# Autodesk Inventor assembly: AssemblyPeleCarotte
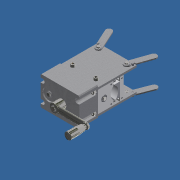
[picture p0: Inventor's stored thumbnail of the model, 180x180]
Saved by Autodesk Inventor 2018 (Build 220112000, 112)
## iProperties
Created: 2022-02-21
Part Number: AssemblyPeleCarotte
Document SubType Name: Assembly
Designer: Nathann
Mass: 1273.76 g
Surface Area: 2275.54 cm^2
Volume: 544.926 cm^3
Density: 2.3375 g/cm^3
Author: Nathann
## Documents named in this file (28)
- C:\Users\Nathann\OneDrive\Objet3D\EPFLEplucheCarrote\V9\AssemblyPeleCarotte-SURFACE-NAT.iam
- C:\Users\Nathann\OneDrive\Objet3D\EPFLEplucheCarrote\V9\Carrot_Peeler_Blade.ipt
- C:\Users\Nathann\OneDrive\Objet3D\EPFLEplucheCarrote\V9\GuideCarotte.ipt
- C:\Users\Nathann\OneDrive\Objet3D\EPFLEplucheCarrote\V9\PlaqueGuideBlocLame.ipt
- C:\Users\Nathann\OneDrive\Objet3D\EPFLEplucheCarrote\V9\2662N415_20DegreePressureAnglePlasticGear.ipt
- C:\Users\Nathann\OneDrive\Objet3D\EPFLEplucheCarrote\V9\2810N4_PlasticMiterGear.ipt
- C:\Users\Nathann\OneDrive\Objet3D\EPFLEplucheCarrote\V9\2662N435_20DegreePressureAnglePlasticGear.ipt
- C:\Users\Nathann\OneDrive\Objet3D\EPFLEplucheCarrote\V9\JointTorique.ipt
- C:\Users\Nathann\Documents\Inventor\Content Center Files\R2018\en-US\SS-ISO 4762\ISO 4762 - M6 x 12SS-ISO.ipt
- C:\Users\Nathann\OneDrive\Objet3D\EPFLEplucheCarrote\V9\Jambe.ipt
- C:\Users\Nathann\OneDrive\Objet3D\EPFLEplucheCarrote\V9\57785K318_Food Industry Dry-Running Sleeve Bearing.ipt
- C:\Users\Nathann\OneDrive\Objet3D\EPFLEplucheCarrote\V9\57785K314_Food Industry Dry-Running Sleeve Bearing-MINOUCHE.ipt
- C:\Users\Nathann\OneDrive\Objet3D\EPFLEplucheCarrote\V9\Roller.ipt
- C:\Users\Nathann\OneDrive\Objet3D\EPFLEplucheCarrote\V9\CarterEngrennage.ipt
- C:\Users\Nathann\OneDrive\Objet3D\EPFLEplucheCarrote\V9\AxeVerticalCaptif.ipt
- C:\Users\Nathann\OneDrive\Objet3D\EPFLEplucheCarrote\V9\AxeVerticalManivelle.ipt
- C:\Users\Nathann\OneDrive\Objet3D\EPFLEplucheCarrote\V9\AxeJambe.ipt
- C:\Users\Nathann\OneDrive\Objet3D\EPFLEplucheCarrote\V9\AxeHorizontalRoller.ipt
- C:\Users\Nathann\OneDrive\Objet3D\EPFLEplucheCarrote\V9\92605A528_Stainless Steel Flat-Tip Set Screw.ipt
- C:\Users\Nathann\OneDrive\Objet3D\EPFLEplucheCarrote\V9\6545N13_303 Stainless Steel Unthreaded Through-Hole Crank Handle.ipt
- C:\Users\Nathann\OneDrive\Objet3D\EPFLEplucheCarrote\V9\2977N13_Rounded Machine Key.ipt
- C:\Users\Nathann\OneDrive\Objet3D\EPFLEplucheCarrote\V9\2977N12_Rounded Machine Key.ipt
- C:\Users\Nathann\OneDrive\Objet3D\EPFLEplucheCarrote\V9\1942N55_Corrosion-Resistant Extension Springs with Hook Ends.ipt
- C:\Users\Nathann\OneDrive\Objet3D\EPFLEplucheCarrote\V9\SupportGuideCarotte.ipt
- C:\Users\Nathann\OneDrive\Objet3D\EPFLEplucheCarrote\V9\93600A511_316 Stainless Steel Dowel Pin.ipt
- C:\Users\Nathann\OneDrive\Objet3D\EPFLEplucheCarrote\V9\93600A531_316 Stainless Steel Dowel Pin.ipt
- C:\Users\Nathann\OneDrive\Objet3D\EPFLEplucheCarrote\V9\98317A224_Side-Mount External Retaining Ring.ipt
- C:\Users\Nathann\OneDrive\Objet3D\EPFLEplucheCarrote\V9\CarterRouleau.ipt
## Components (86 placed, 27 different names)
1. CarterRouleau:1 — Insert:163, Insert:164, Insert:165, Insert:166, Insert:167, Insert:168, Mate:11, Insert:169, Insert:170, Insert:175, Insert:176, Insert:177, Insert:179
2. CarterEngrennage:1 — Insert:21, Insert:22, Insert:23, Insert:24, Insert:85, Insert:93, Insert:97, Insert:98, Insert:167, Insert:168
3. GuideCarotte:1 — Insert:182
4. Carrot_Peeler_Blade:3
5. PlaqueGuideBlocLame:1 — Insert:18, Insert:20, Insert:42, Insert:52, Insert:53, Insert:61, Insert:71, Mate:10, Flush:1, Insert:147, Insert:148, Mate:11, Insert:169, Insert:170, Insert:171, Insert:172
6. PlaqueGuideBlocLame:3 — Insert:104, Insert:119, Insert:120, Insert:145, Insert:146, Insert:177, Insert:178, Insert:179, Insert:180, Insert:181
7. 2662N415_20DegreePressureAnglePlasticGear:1 — Insert:89, Rotation:10, Mate:20, Insert:189, Rotation:17
8. 2810N4_PlasticMiterGear:1 — Insert:83, Mate:19
9. 2810N4_PlasticMiterGear:2 — Insert:89, Rotation:17
10. 2662N435_20DegreePressureAnglePlasticGear:1 — Insert:100, Rotation:2
11. Roller:1 — Insert:82, Insert:83, Mate:18
12. AxeVerticalCaptif:1 — Rotation:4, Rotation:10, Mate:6, Mate:7, Rotation:16, Insert:150, Insert:152, Insert:174, Insert:186, Insert:187, Mate:21, Insert:188
13. AxeVerticalManivelle:1 — Rotation:2, Rotation:4, Mate:2, Mate:3, Mate:4, Mate:5, Rotation:15, Insert:149, Insert:151, Mate:12, Mate:13, Insert:183, Insert:190
14. AxeHorizontalRoller:1 — Insert:81, Mate:8, Mate:9, Rotation:16, Insert:153, Insert:154, Mate:14, Mate:15, Mate:16, Mate:17, Insert:184, Insert:185
15. AxeJambe:1 — Insert:157, Insert:181
16. AxeJambe:2 — Insert:52, Insert:155
17. AxeJambe:3 — Insert:53, Insert:156
18. AxeJambe:4 — Insert:158, Insert:180
19. Jambe:1 — Insert:42, Insert:61
20. Jambe:3 — Insert:120
21. Jambe:4 — Insert:119
22. Jambe:5 — Insert:71
23. 57785K318_Food Industry Dry-Running Sleeve Bearing:1 — Insert:93, Insert:138
24. 57785K318_Food Industry Dry-Running Sleeve Bearing:2 — Insert:98, Insert:100
25. 57785K314_Food Industry Dry-Running Sleeve Bearing-MINOUCHE:1 — Insert:82, Insert:176
26. 57785K314_Food Industry Dry-Running Sleeve Bearing-MINOUCHE:2
27. 57785K314_Food Industry Dry-Running Sleeve Bearing-MINOUCHE:4 — Insert:97, Insert:189
28. 57785K314_Food Industry Dry-Running Sleeve Bearing-MINOUCHE:5 — Insert:81, Insert:175, Insert:185
29. 57785K314_Food Industry Dry-Running Sleeve Bearing-MINOUCHE:6 — Insert:85, Insert:174, Insert:187
30. SupportGuideCarotte:1 — Insert:141, Insert:142, Mate:10, Flush:1, Insert:159, Insert:160, Insert:161, Insert:162, Insert:182
31. 6545N13_303 Stainless Steel Unthreaded Through-Hole Crank Handle:1 — Insert:138, Rotation:15, Insert:183
32. JointTorique:10
33. JointTorique:11
34. JointTorique:12
35. JointTorique:13
36. JointTorique:14
37. JointTorique:15
38. JointTorique:16
39. JointTorique:17
40. 92605A528_Stainless Steel Flat-Tip Set Screw:1
41. 92605A528_Stainless Steel Flat-Tip Set Screw:2
42. 2977N13_Rounded Machine Key:1 — Mate:4, Mate:5, Insert:190
43. 2977N13_Rounded Machine Key:2 — Mate:2, Mate:3, Mate:12, Mate:13
44. 2977N12_Rounded Machine Key:2 — Mate:6, Mate:7, Mate:20, Mate:21, Insert:188
45. 2977N12_Rounded Machine Key:4 — Mate:8, Mate:9, Mate:14, Mate:16
46. 1942N55_Corrosion-Resistant Extension Springs with Hook Ends:1
47. 1942N55_Corrosion-Resistant Extension Springs with Hook Ends:2
48. 1942N55_Corrosion-Resistant Extension Springs with Hook Ends:3
49. 1942N55_Corrosion-Resistant Extension Springs with Hook Ends:4
50. 1942N55_Corrosion-Resistant Extension Springs with Hook Ends:5
51. 1942N55_Corrosion-Resistant Extension Springs with Hook Ends:6
52. 1942N55_Corrosion-Resistant Extension Springs with Hook Ends:7
53. 1942N55_Corrosion-Resistant Extension Springs with Hook Ends:8
54. 93600A511_316 Stainless Steel Dowel Pin:1 — Insert:146
55. 93600A531_316 Stainless Steel Dowel Pin:1 — Insert:163
56. 93600A511_316 Stainless Steel Dowel Pin:2 — Insert:145
57. 93600A511_316 Stainless Steel Dowel Pin:3 — Insert:147
58. 93600A511_316 Stainless Steel Dowel Pin:4 — Insert:148
59. 93600A531_316 Stainless Steel Dowel Pin:2 — Insert:164
60. 93600A531_316 Stainless Steel Dowel Pin:3 — Insert:165
61. 93600A531_316 Stainless Steel Dowel Pin:4 — Insert:166
62. 93600A531_316 Stainless Steel Dowel Pin:5 — Insert:162
63. 93600A531_316 Stainless Steel Dowel Pin:6 — Insert:161
64. 93600A531_316 Stainless Steel Dowel Pin:7 — Insert:159
65. 93600A531_316 Stainless Steel Dowel Pin:8 — Insert:160
66. 98317A224_Side-Mount External Retaining Ring:1 — Insert:149
67. 98317A224_Side-Mount External Retaining Ring:2 — Insert:150, Insert:186
68. 98317A224_Side-Mount External Retaining Ring:3 — Insert:154, Insert:184
69. 98317A224_Side-Mount External Retaining Ring:4 — Insert:151
70. 98317A224_Side-Mount External Retaining Ring:5 — Insert:152
71. 98317A224_Side-Mount External Retaining Ring:6 — Insert:153
72. 98317A224_Side-Mount External Retaining Ring:7 — Insert:157
73. 98317A224_Side-Mount External Retaining Ring:8 — Insert:158
74. 98317A224_Side-Mount External Retaining Ring:9 — Insert:156
75. 98317A224_Side-Mount External Retaining Ring:10 — Insert:155
76. SS ISO 4762 M6 x 12:4 — Insert:141
77. SS ISO 4762 M6 x 12:5 — Insert:178
78. SS ISO 4762 M6 x 12:6 — Insert:104
79. SS ISO 4762 M6 x 12:8 — Insert:18, Insert:171
80. SS ISO 4762 M6 x 12:10 — Insert:22
81. SS ISO 4762 M6 x 12:11 — Insert:20, Insert:172
82. SS ISO 4762 M6 x 12:12 — Insert:23
83. SS ISO 4762 M6 x 12:13 — Insert:24
84. SS ISO 4762 M6 x 12:14 — Insert:21
85. SS ISO 4762 M6 x 12:15 — Insert:142
86. 2977N12_Rounded Machine Key:5 — Mate:15, Mate:17, Mate:18, Mate:19
## Relationships (98: Insert 71, Mate 20, RelateRotation 6, Flush 1)
- Insert:18: PlaqueGuideBlocLame:1 ↔ SS ISO 4762 M6 x 12:8
- Insert:20: PlaqueGuideBlocLame:1 ↔ SS ISO 4762 M6 x 12:11
- Insert:21: CarterEngrennage:1 ↔ SS ISO 4762 M6 x 12:14
- Insert:22: CarterEngrennage:1 ↔ SS ISO 4762 M6 x 12:10
- Insert:23: CarterEngrennage:1 ↔ SS ISO 4762 M6 x 12:12
- Insert:24: CarterEngrennage:1 ↔ SS ISO 4762 M6 x 12:13
- Insert:42: PlaqueGuideBlocLame:1 ↔ Jambe:1
- Insert:52: PlaqueGuideBlocLame:1 ↔ AxeJambe:2
- Insert:53: PlaqueGuideBlocLame:1 ↔ AxeJambe:3
- Insert:61: PlaqueGuideBlocLame:1 ↔ Jambe:1
- Insert:71: PlaqueGuideBlocLame:1 ↔ Jambe:5
- Insert:81: AxeHorizontalRoller:1 ↔ 57785K314_Food Industry Dry-Running Sleeve Bearing-MINOUCHE:5
- Insert:82: Roller:1 ↔ 57785K314_Food Industry Dry-Running Sleeve Bearing-MINOUCHE:1
- Insert:83: 2810N4_PlasticMiterGear:1 ↔ Roller:1
- Insert:85: CarterEngrennage:1 ↔ 57785K314_Food Industry Dry-Running Sleeve Bearing-MINOUCHE:6
- Insert:89: 2662N415_20DegreePressureAnglePlasticGear:1 ↔ 2810N4_PlasticMiterGear:2
- Insert:93: CarterEngrennage:1 ↔ 57785K318_Food Industry Dry-Running Sleeve Bearing:1
- Insert:97: CarterEngrennage:1 ↔ 57785K314_Food Industry Dry-Running Sleeve Bearing-MINOUCHE:4
- Insert:98: CarterEngrennage:1 ↔ 57785K318_Food Industry Dry-Running Sleeve Bearing:2
- Insert:100: 2662N435_20DegreePressureAnglePlasticGear:1 ↔ 57785K318_Food Industry Dry-Running Sleeve Bearing:2
- Rotation:2 [RelateRotation] (1 ul): 2662N435_20DegreePressureAnglePlasticGear:1 ↔ AxeVerticalManivelle:1
- Rotation:4 [RelateRotation] (0.25 ul): AxeVerticalCaptif:1 ↔ AxeVerticalManivelle:1
- Rotation:10 [RelateRotation] (-1 ul): 2662N415_20DegreePressureAnglePlasticGear:1 ↔ AxeVerticalCaptif:1
- Insert:104: PlaqueGuideBlocLame:3 ↔ SS ISO 4762 M6 x 12:6
- Insert:119: PlaqueGuideBlocLame:3 ↔ Jambe:4
- Insert:120: PlaqueGuideBlocLame:3 ↔ Jambe:3
- Mate:2: AxeVerticalManivelle:1 ↔ 2977N13_Rounded Machine Key:2
- Mate:3: AxeVerticalManivelle:1 ↔ 2977N13_Rounded Machine Key:2
- Mate:4: AxeVerticalManivelle:1 ↔ 2977N13_Rounded Machine Key:1
- Mate:5: AxeVerticalManivelle:1 ↔ 2977N13_Rounded Machine Key:1
- Insert:138: 57785K318_Food Industry Dry-Running Sleeve Bearing:1 ↔ 6545N13_303 Stainless Steel Unthreaded Through-Hole Crank Handle:1
- Rotation:15 [RelateRotation] (-1 ul): AxeVerticalManivelle:1 ↔ 6545N13_303 Stainless Steel Unthreaded Through-Hole Crank Handle:1
- Mate:6: AxeVerticalCaptif:1 ↔ 2977N12_Rounded Machine Key:2
- Mate:7: AxeVerticalCaptif:1 ↔ 2977N12_Rounded Machine Key:2
- Mate:8: AxeHorizontalRoller:1 ↔ 2977N12_Rounded Machine Key:4
- Mate:9: AxeHorizontalRoller:1 ↔ 2977N12_Rounded Machine Key:4
- Rotation:16 [RelateRotation] (1 ul): AxeVerticalCaptif:1 ↔ AxeHorizontalRoller:1
- Insert:141: SupportGuideCarotte:1 ↔ SS ISO 4762 M6 x 12:4
- Insert:142: SupportGuideCarotte:1 ↔ SS ISO 4762 M6 x 12:15
- Mate:10: PlaqueGuideBlocLame:1 ↔ SupportGuideCarotte:1
- Flush:1: PlaqueGuideBlocLame:1 ↔ SupportGuideCarotte:1
- Insert:145: PlaqueGuideBlocLame:3 ↔ 93600A511_316 Stainless Steel Dowel Pin:2
- Insert:146: PlaqueGuideBlocLame:3 ↔ 93600A511_316 Stainless Steel Dowel Pin:1
- Insert:147: PlaqueGuideBlocLame:1 ↔ 93600A511_316 Stainless Steel Dowel Pin:3
- Insert:148: PlaqueGuideBlocLame:1 ↔ 93600A511_316 Stainless Steel Dowel Pin:4
- Insert:149: AxeVerticalManivelle:1 ↔ 98317A224_Side-Mount External Retaining Ring:1
- Insert:150: AxeVerticalCaptif:1 ↔ 98317A224_Side-Mount External Retaining Ring:2
- Insert:151: AxeVerticalManivelle:1 ↔ 98317A224_Side-Mount External Retaining Ring:4
- Insert:152: AxeVerticalCaptif:1 ↔ 98317A224_Side-Mount External Retaining Ring:5
- Insert:153: AxeHorizontalRoller:1 ↔ 98317A224_Side-Mount External Retaining Ring:6
- Insert:154: AxeHorizontalRoller:1 ↔ 98317A224_Side-Mount External Retaining Ring:3
- Insert:155: AxeJambe:2 ↔ 98317A224_Side-Mount External Retaining Ring:10
- Insert:156: AxeJambe:3 ↔ 98317A224_Side-Mount External Retaining Ring:9
- Insert:157: AxeJambe:1 ↔ 98317A224_Side-Mount External Retaining Ring:7
- Insert:158: AxeJambe:4 ↔ 98317A224_Side-Mount External Retaining Ring:8
- Insert:159: SupportGuideCarotte:1 ↔ 93600A531_316 Stainless Steel Dowel Pin:7
- Insert:160: SupportGuideCarotte:1 ↔ 93600A531_316 Stainless Steel Dowel Pin:8
- Insert:161: SupportGuideCarotte:1 ↔ 93600A531_316 Stainless Steel Dowel Pin:6
- Insert:162: SupportGuideCarotte:1 ↔ 93600A531_316 Stainless Steel Dowel Pin:5
- Insert:163: CarterRouleau:1 ↔ 93600A531_316 Stainless Steel Dowel Pin:1
- Insert:164: CarterRouleau:1 ↔ 93600A531_316 Stainless Steel Dowel Pin:2
- Insert:165: CarterRouleau:1 ↔ 93600A531_316 Stainless Steel Dowel Pin:3
- Insert:166: CarterRouleau:1 ↔ 93600A531_316 Stainless Steel Dowel Pin:4
- Insert:167: CarterRouleau:1 ↔ CarterEngrennage:1
- Insert:168: CarterRouleau:1 ↔ CarterEngrennage:1
- Mate:11: CarterRouleau:1 ↔ PlaqueGuideBlocLame:1
- Insert:169: CarterRouleau:1 ↔ PlaqueGuideBlocLame:1
- Insert:170: CarterRouleau:1 ↔ PlaqueGuideBlocLame:1
- Insert:171: PlaqueGuideBlocLame:1 ↔ SS ISO 4762 M6 x 12:8
- Insert:172: PlaqueGuideBlocLame:1 ↔ SS ISO 4762 M6 x 12:11
- Insert:174: AxeVerticalCaptif:1 ↔ 57785K314_Food Industry Dry-Running Sleeve Bearing-MINOUCHE:6
- Insert:175: CarterRouleau:1 ↔ 57785K314_Food Industry Dry-Running Sleeve Bearing-MINOUCHE:5
- Insert:176: CarterRouleau:1 ↔ 57785K314_Food Industry Dry-Running Sleeve Bearing-MINOUCHE:1
- Insert:177: CarterRouleau:1 ↔ PlaqueGuideBlocLame:3
- Insert:178: PlaqueGuideBlocLame:3 ↔ SS ISO 4762 M6 x 12:5
- Insert:179: CarterRouleau:1 ↔ PlaqueGuideBlocLame:3
- Insert:180: PlaqueGuideBlocLame:3 ↔ AxeJambe:4
- Insert:181: PlaqueGuideBlocLame:3 ↔ AxeJambe:1
- Insert:182: GuideCarotte:1 ↔ SupportGuideCarotte:1
- Mate:12: AxeVerticalManivelle:1 ↔ 2977N13_Rounded Machine Key:2
- Mate:13: AxeVerticalManivelle:1 ↔ 2977N13_Rounded Machine Key:2
- Insert:183: AxeVerticalManivelle:1 ↔ 6545N13_303 Stainless Steel Unthreaded Through-Hole Crank Handle:1
- Mate:14: AxeHorizontalRoller:1 ↔ 2977N12_Rounded Machine Key:4
- Mate:15: AxeHorizontalRoller:1 ↔ 2977N12_Rounded Machine Key:5
- Mate:16: AxeHorizontalRoller:1 ↔ 2977N12_Rounded Machine Key:4
- Mate:17: AxeHorizontalRoller:1 ↔ 2977N12_Rounded Machine Key:5
- Insert:184: AxeHorizontalRoller:1 ↔ 98317A224_Side-Mount External Retaining Ring:3
- Insert:185: AxeHorizontalRoller:1 ↔ 57785K314_Food Industry Dry-Running Sleeve Bearing-MINOUCHE:5
- Mate:18: Roller:1 ↔ 2977N12_Rounded Machine Key:5
- Mate:19: 2810N4_PlasticMiterGear:1 ↔ 2977N12_Rounded Machine Key:5
- Insert:186: AxeVerticalCaptif:1 ↔ 98317A224_Side-Mount External Retaining Ring:2
- Insert:187: AxeVerticalCaptif:1 ↔ 57785K314_Food Industry Dry-Running Sleeve Bearing-MINOUCHE:6
- Mate:20: 2662N415_20DegreePressureAnglePlasticGear:1 ↔ 2977N12_Rounded Machine Key:2
- Mate:21: AxeVerticalCaptif:1 ↔ 2977N12_Rounded Machine Key:2
- Insert:188: AxeVerticalCaptif:1 ↔ 2977N12_Rounded Machine Key:2
- Insert:189: 2662N415_20DegreePressureAnglePlasticGear:1 ↔ 57785K314_Food Industry Dry-Running Sleeve Bearing-MINOUCHE:4
- Insert:190: AxeVerticalManivelle:1 ↔ 2977N13_Rounded Machine Key:1
- Rotation:17 [RelateRotation] (1 ul): 2662N415_20DegreePressureAnglePlasticGear:1 ↔ 2810N4_PlasticMiterGear:2
